# Autodesk Inventor assembly: robot
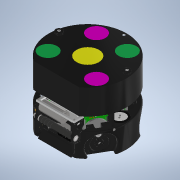
[picture p0: Inventor's stored thumbnail of the model, 180x180]
Saved by Autodesk Inventor 2020.4 (Build 244396000, 396)
## iProperties
Created: 2021-05-09
Part Number: robot
Document SubType Name: Assembly
Designer: Acer
Author: Acer
## Documents named in this file (7)
- C:\Users\Acer\Documents\MATLAB\Doutorado\CAD\Inventor\robot.iam
- C:\Users\Acer\Documents\MATLAB\Doutorado\CAD\Inventor\first_floor\first_floor.iam
- C:\Users\Acer\Documents\MATLAB\Doutorado\CAD\Inventor\other\grass.ipt
- C:\Users\Acer\Documents\MATLAB\Doutorado\CAD\Inventor\other\Golfball.ipt
- C:\Users\Acer\Documents\MATLAB\Doutorado\CAD\Inventor\first_floor\Kicker\kicker_assembly.iam
- C:\Users\Acer\Documents\MATLAB\Doutorado\CAD\Inventor\sec_floor\sec_floor.iam
- C:\Users\Acer\Documents\Inventor\Content Center Files\R2020\en-US\DIN 84\DIN 84 - M3 x 10.ipt
## Components (9 placed, 6 different names)
1. first_floor:1 [sub-assembly] — Mate:1, Flush:1, Flush:2, Tangent:2, Mate:2, Mate:3, Mate:4, Mate:5, Angle:1, Mate:6, Mate:7, Mate:8, Mate:9, Mate:10, Mate:11, Mate:12, Mate:13, Mate:14
2. grass:1 — Mate:1, Flush:1, Flush:2, Tangent:1
3. Golfball:1 — Tangent:1, Tangent:2
4. Kicker Assembly:1 [sub-assembly] — Mate:2, Mate:3, Mate:4
5. sec_floor:1 [sub-assembly] — Mate:5, Angle:1, Mate:6
6. DIN 84 - replaced by DIN EN ISO 1207 M3 x 10:1 — Mate:7, Mate:13
7. DIN 84 - replaced by DIN EN ISO 1207 M3 x 10:2 — Mate:8, Mate:12
8. DIN 84 - replaced by DIN EN ISO 1207 M3 x 10:3 — Mate:9, Mate:11
9. DIN 84 - replaced by DIN EN ISO 1207 M3 x 10:4 — Mate:10, Mate:14
## Relationships (19: Mate 14, Flush 2, Tangent 2, Angle 1)
- Mate:1 (4 mm): first_floor:1 ↔ grass:1
- Flush:1 (-200 mm): first_floor:1 ↔ grass:1
- Flush:2 (-110 mm): first_floor:1 ↔ grass:1
- Tangent:1: grass:1 ↔ Golfball:1
- Tangent:2: first_floor:1 ↔ Golfball:1
- Mate:2: first_floor:1 ↔ Kicker Assembly:1
- Mate:3: first_floor:1 ↔ Kicker Assembly:1
- Mate:4: first_floor:1 ↔ Kicker Assembly:1
- Mate:5: first_floor:1 ↔ sec_floor:1
- Angle:1 (0 deg): first_floor:1 ↔ sec_floor:1
- Mate:6 (0.1 mm): first_floor:1 ↔ sec_floor:1
- Mate:7: first_floor:1 ↔ DIN 84 - replaced by DIN EN ISO 1207 M3 x 10:1
- Mate:8: first_floor:1 ↔ DIN 84 - replaced by DIN EN ISO 1207 M3 x 10:2
- Mate:9: first_floor:1 ↔ DIN 84 - replaced by DIN EN ISO 1207 M3 x 10:3
- Mate:10: first_floor:1 ↔ DIN 84 - replaced by DIN EN ISO 1207 M3 x 10:4
- Mate:11: first_floor:1 ↔ DIN 84 - replaced by DIN EN ISO 1207 M3 x 10:3
- Mate:12: first_floor:1 ↔ DIN 84 - replaced by DIN EN ISO 1207 M3 x 10:2
- Mate:13: first_floor:1 ↔ DIN 84 - replaced by DIN EN ISO 1207 M3 x 10:1
- Mate:14: first_floor:1 ↔ DIN 84 - replaced by DIN EN ISO 1207 M3 x 10:4
